# Autodesk Inventor assembly: GUS
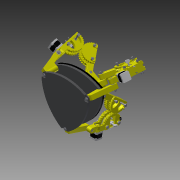
[picture p0: Inventor's stored thumbnail of the model, 180x180]
Saved by Autodesk Inventor 2013 (Build 170138000, 138)
## iProperties
Created: 2013-11-26
Part Number: GUS
Document SubType Name: Assembly
Designer: employee
d13: 0.000 mm
Author: employee
## Documents named in this file (16)
- C:\Users\employee\Desktop\GUS Simpson\GUS.iam
- C:\Users\employee\Desktop\GUS Simpson\_BASALT BED.ipt
- C:\Users\employee\Desktop\GUS Simpson\_BOTTOM PLATE.ipt
- C:\Users\employee\Desktop\GUS Simpson\_TOP PLATE.ipt
- C:\Users\employee\Desktop\GUS Simpson\SHOULDER.iam
- C:\Users\employee\Desktop\GUS Simpson\M8x100.ipt
- C:\Users\employee\Desktop\GUS Simpson\PLASTIC WASHER.ipt
- C:\Users\employee\Desktop\GUS Simpson\M8 NUT.ipt
- C:\Users\employee\Desktop\GUS Simpson\MOTOR ARM.iam
- C:\Users\employee\Desktop\GUS Simpson\HUB BOTTOM.iam
- C:\Users\employee\Desktop\GUS Simpson\HUB CENTER.iam
- C:\Users\employee\Desktop\GUS Simpson\HUB TOP.iam
- C:\Users\employee\Desktop\GUS Simpson\M4 NUT.ipt
- C:\Users\employee\Desktop\GUS Simpson\LOCK NUT.ipt
- C:\Users\employee\Desktop\GUS Simpson\BOWDEN NUT.ipt
- C:\Users\employee\Desktop\GUS Simpson\SLAVE ARM.iam
## Components (27 placed, 15 different names)
1. _BASALT BED:1 — Mate:1, Flush:1, Flush:2, Insert:1, Insert:2, Insert:8, Insert:9, Insert:10
2. _BOTTOM PLATE:1 — Insert:6, Insert:7, Insert:14, Insert:15, Insert:16
3. _TOP PLATE:1 — Insert:1, Insert:2, Insert:3, Insert:4, Insert:5
4. SHOULDER:1 [sub-assembly] — Insert:3, Insert:7, Insert:17, Mate:5
5. SHOULDER:2 [sub-assembly] — Insert:4, Insert:19, Mate:6
6. SHOULDER:3 [sub-assembly] — Insert:5, Insert:6, Insert:18
7. M8x100:1 — Insert:11, Angle:2
8. M8x100:2 — Insert:12, Angle:3
9. M8x100:3 — Insert:13, Angle:1
10. PLASTIC WASHER:1 — Insert:8, Insert:11
11. PLASTIC WASHER:2 — Insert:10, Insert:13
12. PLASTIC WASHER:3 — Insert:9, Insert:12
13. M8 NUT:1 — Insert:14, Angle:6
14. M8 NUT:2 — Insert:15, Angle:5
15. M8 NUT:3 — Insert:16, Angle:4
16. MOTOR ARM:1 [sub-assembly] — Insert:19, Flush:4, Mate:3, Mate:9
17. MOTOR ARM:2 [sub-assembly] — Insert:18, Flush:5, Mate:4, Mate:7, Mate:10
18. MOTOR ARM:3 [sub-assembly] — Insert:17, Mate:2, Flush:3, Mate:8
19. HUB BOTTOM:1 [sub-assembly] — Insert:20, Insert:22, Angle:7, Angle:8, Angle:9, Insert:26, Mate:6
20. HUB CENTER:1 [sub-assembly] — Insert:20, Insert:21, Insert:27, Mate:5
21. HUB TOP:1 [sub-assembly] — Insert:21, Insert:23, Insert:25
22. M4 NUT:1 — Insert:22, Angle:7, Insert:24
23. LOCK NUT:1 — Insert:23, Angle:8
24. BOWDEN NUT:1 — Insert:24, Angle:9
25. SLAVE ARM:1 [sub-assembly] — Insert:27, Mate:2, Flush:3, Mate:8
26. SLAVE ARM:2 [sub-assembly] — Insert:26, Flush:4, Mate:3, Mate:9
27. SLAVE ARM:3 [sub-assembly] — Insert:25, Flush:5, Mate:4, Mate:7, Mate:10
## Relationships (51: Insert 27, Mate 10, Angle 9, Flush 5)
- Mate:1: _BASALT BED:1
- Flush:1: _BASALT BED:1
- Flush:2: _BASALT BED:1
- Insert:1: _BASALT BED:1 ↔ _TOP PLATE:1
- Insert:2: _BASALT BED:1 ↔ _TOP PLATE:1
- Insert:3: _TOP PLATE:1 ↔ SHOULDER:1
- Insert:4: _TOP PLATE:1 ↔ SHOULDER:2
- Insert:5: _TOP PLATE:1 ↔ SHOULDER:3
- Insert:6: _BOTTOM PLATE:1 ↔ SHOULDER:3
- Insert:7: _BOTTOM PLATE:1 ↔ SHOULDER:1
- Insert:8: _BASALT BED:1 ↔ PLASTIC WASHER:1
- Insert:9: _BASALT BED:1 ↔ PLASTIC WASHER:3
- Insert:10: _BASALT BED:1 ↔ PLASTIC WASHER:2
- Insert:11: M8x100:1 ↔ PLASTIC WASHER:1
- Insert:12: M8x100:2 ↔ PLASTIC WASHER:3
- Insert:13: M8x100:3 ↔ PLASTIC WASHER:2
- Angle:1 (0 deg): M8x100:3
- Angle:2 (0 deg): M8x100:1
- Angle:3 (0 deg): M8x100:2
- Insert:14: _BOTTOM PLATE:1 ↔ M8 NUT:1
- Insert:15: _BOTTOM PLATE:1 ↔ M8 NUT:2
- Insert:16: _BOTTOM PLATE:1 ↔ M8 NUT:3
- Angle:4 (0 deg): M8 NUT:3
- Angle:5 (0 deg): M8 NUT:2
- Angle:6 (0 deg): M8 NUT:1
- Insert:17: SHOULDER:1 ↔ MOTOR ARM:3
- Insert:18: SHOULDER:3 ↔ MOTOR ARM:2
- Insert:19: SHOULDER:2 ↔ MOTOR ARM:1
- Insert:20: HUB BOTTOM:1 ↔ HUB CENTER:1
- Insert:21: HUB CENTER:1 ↔ HUB TOP:1
- Insert:22: HUB BOTTOM:1 ↔ M4 NUT:1
- Angle:7 (0 deg): HUB BOTTOM:1 ↔ M4 NUT:1
- Insert:23: HUB TOP:1 ↔ LOCK NUT:1
- Angle:8 (0 deg): HUB BOTTOM:1 ↔ LOCK NUT:1
- Insert:24: M4 NUT:1 ↔ BOWDEN NUT:1
- Angle:9 (30 deg): HUB BOTTOM:1 ↔ BOWDEN NUT:1
- Insert:25: HUB TOP:1 ↔ SLAVE ARM:3
- Insert:26: HUB BOTTOM:1 ↔ SLAVE ARM:2
- Insert:27: HUB CENTER:1 ↔ SLAVE ARM:1
- Mate:2 (100 mm): MOTOR ARM:3 ↔ SLAVE ARM:1
- Flush:3: MOTOR ARM:3 ↔ SLAVE ARM:1
- Flush:4: MOTOR ARM:1 ↔ SLAVE ARM:2
- Mate:3 (100 mm): MOTOR ARM:1 ↔ SLAVE ARM:2
- Flush:5: MOTOR ARM:2 ↔ SLAVE ARM:3
- Mate:4 (100 mm): MOTOR ARM:2 ↔ SLAVE ARM:3
- Mate:5 (159.3691 mm): SHOULDER:1 ↔ HUB CENTER:1
- Mate:6 (159.3691 mm): SHOULDER:2 ↔ HUB BOTTOM:1
- Mate:7 (159.3691 mm): MOTOR ARM:2 ↔ SLAVE ARM:3
- Mate:8 (118.4704 mm): MOTOR ARM:3 ↔ SLAVE ARM:1
- Mate:9 (118.4704 mm): MOTOR ARM:1 ↔ SLAVE ARM:2
- Mate:10 (118.4704 mm): MOTOR ARM:2 ↔ SLAVE ARM:3
## Named parameters: x = 0 mm, y = 0 mm, z = 0 mm, l1 = 125 mm, l2 = 72.16878 mm, m1 = 159.36906 mm, m2 = 159.36906 mm, m3 = 159.36906 mm, d = 67.566 mm
